# Autodesk Inventor assembly: Assembly-RoundBreadboard_V2
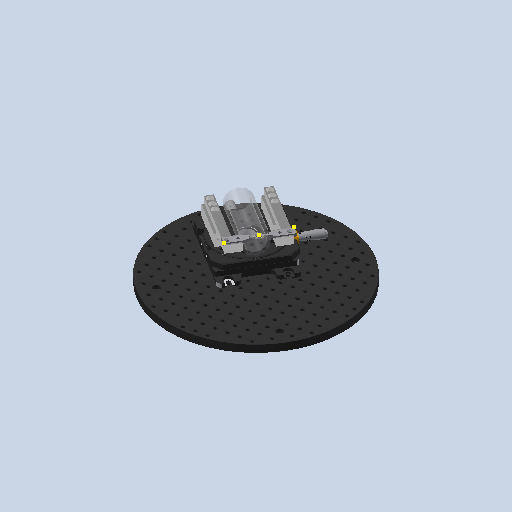
[picture p0: Inventor's stored thumbnail of the model, 512x512]
Saved by Autodesk Inventor 2022 (Build 260153000, 153)
## iProperties
Created: 2016-10-31
Part Number: Assembly-RoundBreadboard_V2
Document SubType Name: Assembly
Designer: Eivind
Author: Eivind
## Documents named in this file (9)
- E:\Dropbox (UIO Physiology Dropbox)\Lab Data\Eivind Hennestad\Projects\AHV\Setup\Inventor Project\Assembly-RotatablePlatform.iam
- E:\Dropbox (UIO Physiology Dropbox)\Lab Data\Eivind Hennestad\Projects\AHV\Setup\Inventor Project\Parts - PortableRotationStage\Thorlabs-MBR300_M-BreadboardRound300mm.ipt
- E:\Dropbox (UIO Physiology Dropbox)\Lab Data\Eivind Hennestad\Projects\AHV\Setup\Inventor Project\Parts - PortableRotationStage\Thorlabs-XYR-M.ipt
- E:\Dropbox (UIO Physiology Dropbox)\Lab Data\Eivind Hennestad\Projects\AHV\Setup\Inventor Project\Parts - PortableRotationStage\Custom-PlexiTubeAnimal.ipt
- E:\Dropbox (UIO Physiology Dropbox)\Lab Data\Eivind Hennestad\Projects\AHV\Setup\Inventor Project\Parts - HeadbarFixation\Custom-Headbar-OShape.ipt
- E:\Dropbox (UIO Physiology Dropbox)\Lab Data\Eivind Hennestad\Projects\AHV\Setup\Inventor Project\Parts - HeadbarFixation\HeadbarClampBottom.ipt
- E:\Dropbox (UIO Physiology Dropbox)\Lab Data\Eivind Hennestad\Projects\AHV\Setup\Inventor Project\Parts - HeadbarFixation\HeadbarHolderBracketAdjustable20mm.ipt
- E:\Dropbox (UIO Physiology Dropbox)\Lab Data\Eivind Hennestad\Projects\AHV\Setup\Inventor Project\Parts - HeadbarFixation\HeadbarHolder_v2.ipt
- E:\Dropbox (UIO Physiology Dropbox)\Lab Data\Eivind Hennestad\Projects\AHV\Setup\Inventor Project\Parts - HeadbarFixation\HeadbarHolderMirrored_v2.ipt
## Components (10 placed, 8 different names)
1. Thorlabs-MBR300_M-BreadboardRound300mm:1 — Mate:1, Mate:2, Mate:15
2. Thorlabs-XYR-M:1 — Mate:1, Mate:2, Tangent:1, Flush:14, Mate:13, Mate:15, Mate:24, Mate:25, Mate:26, Mate:27, Mate:28, Mate:29, Mate:30
3. HeadbarHolder_v2:1 — Mate:19, Mate:20, Mate:32, Mate:33
4. HeadbarHolderMirrored_v2:1 — Angle:3, Mate:35, Mate:36, Angle:4, Mate:37
5. Custom-PlexiTubeAnimal:1 — Tangent:1, Flush:14, Mate:13
6. Custom-Headbar-OShape:1 — Mate:17, Mate:18, Mate:21, Mate:22, Mate:23, Mate:31
7. HeadbarClampBottom:1 — Angle:3, Mate:17, Mate:18, Mate:31, Mate:37
8. HeadbarClampBottom:2 — Mate:19, Mate:20, Mate:21, Mate:22, Mate:23
9. HeadbarHolderBracketAdjustable20mm:1 — Mate:24, Mate:26, Mate:27, Mate:32, Mate:33
10. HeadbarHolderBracketAdjustable20mm:2 — Mate:25, Mate:28, Mate:29, Mate:30, Mate:35, Mate:36, Angle:4
## Relationships (28: Mate 24, Angle 2, Tangent 1, Flush 1)
- Mate:1: Thorlabs-MBR300_M-BreadboardRound300mm:1 ↔ Thorlabs-XYR-M:1
- Mate:2: Thorlabs-MBR300_M-BreadboardRound300mm:1 ↔ Thorlabs-XYR-M:1
- Tangent:1: Thorlabs-XYR-M:1 ↔ Custom-PlexiTubeAnimal:1
- Flush:14 (15 mm): Thorlabs-XYR-M:1 ↔ Custom-PlexiTubeAnimal:1
- Mate:13: Thorlabs-XYR-M:1 ↔ Custom-PlexiTubeAnimal:1
- Angle:3 (180 deg): HeadbarHolderMirrored_v2:1 ↔ HeadbarClampBottom:1
- Mate:15: Thorlabs-MBR300_M-BreadboardRound300mm:1 ↔ Thorlabs-XYR-M:1
- Mate:17: Custom-Headbar-OShape:1 ↔ HeadbarClampBottom:1
- Mate:18: Custom-Headbar-OShape:1 ↔ HeadbarClampBottom:1
- Mate:19: HeadbarHolder_v2:1 ↔ HeadbarClampBottom:2
- Mate:20 (0.1 mm): HeadbarHolder_v2:1 ↔ HeadbarClampBottom:2
- Mate:21: Custom-Headbar-OShape:1 ↔ HeadbarClampBottom:2
- Mate:22: Custom-Headbar-OShape:1 ↔ HeadbarClampBottom:2
- Mate:23: Custom-Headbar-OShape:1 ↔ HeadbarClampBottom:2
- Mate:24: Thorlabs-XYR-M:1 ↔ HeadbarHolderBracketAdjustable20mm:1
- Mate:25: Thorlabs-XYR-M:1 ↔ HeadbarHolderBracketAdjustable20mm:2
- Mate:26: Thorlabs-XYR-M:1 ↔ HeadbarHolderBracketAdjustable20mm:1
- Mate:27: Thorlabs-XYR-M:1 ↔ HeadbarHolderBracketAdjustable20mm:1
- Mate:28: Thorlabs-XYR-M:1 ↔ HeadbarHolderBracketAdjustable20mm:2
- Mate:29: Thorlabs-XYR-M:1 ↔ HeadbarHolderBracketAdjustable20mm:2
- Mate:30: Thorlabs-XYR-M:1 ↔ HeadbarHolderBracketAdjustable20mm:2
- Mate:31: Custom-Headbar-OShape:1 ↔ HeadbarClampBottom:1
- Mate:32: HeadbarHolder_v2:1 ↔ HeadbarHolderBracketAdjustable20mm:1
- Mate:33: HeadbarHolder_v2:1 ↔ HeadbarHolderBracketAdjustable20mm:1
- Mate:35: HeadbarHolderMirrored_v2:1 ↔ HeadbarHolderBracketAdjustable20mm:2
- Mate:36: HeadbarHolderMirrored_v2:1 ↔ HeadbarHolderBracketAdjustable20mm:2
- Angle:4 (0 deg): HeadbarHolderMirrored_v2:1 ↔ HeadbarHolderBracketAdjustable20mm:2
- Mate:37 (0.1 mm): HeadbarHolderMirrored_v2:1 ↔ HeadbarClampBottom:1
